# Autodesk Inventor assembly: !SCARA assembly
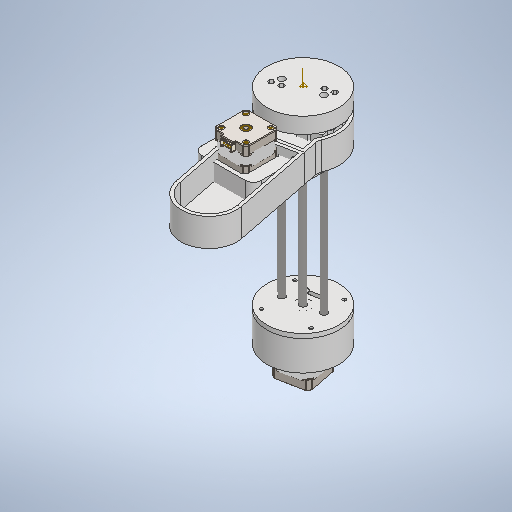
[picture p0: Inventor's stored thumbnail of the model, 512x512]
Saved by Autodesk Inventor 2025.2 (Build 292293000, 293)
## iProperties
Created: 2025-01-25
Part Number: !SCARA assembly
Document SubType Name: Assembly
Designer: caomi
Author: caomi
## Documents named in this file (18)
- C:\Minh Nguyen\H2A\cad\SCARA\!SCARA assembly.iam
- C:\Minh Nguyen\H2A\cad\SCARA\SCARA base.ipt
- C:\Minh Nguyen\H2A\cad\SCARA\Stepper Motor 17HS3401.ipt
- C:\Minh Nguyen\H2A\cad\SCARA\608 Bearing.ipt
- C:\Minh Nguyen\H2A\cad\SCARA\Shaft support.ipt
- C:\Minh Nguyen\H2A\cad\SCARA\SCARA swivel base - bottom.ipt
- C:\Minh Nguyen\H2A\cad\SCARA\Guide rods.ipt
- C:\Minh Nguyen\H2A\cad\SCARA\SCARA swivel base - mid.ipt
- C:\Minh Nguyen\H2A\cad\SCARA\Lead screw.ipt
- C:\Minh Nguyen\H2A\cad\SCARA\SCARA swivel connection rod.ipt
- C:\Minh Nguyen\H2A\cad\SCARA\Bearing block.ipt
- C:\Minh Nguyen\H2A\cad\SCARA\Lead nut.ipt
- C:\Minh Nguyen\H2A\cad\SCARA\SCARA arm base.ipt
- C:\Minh Nguyen\H2A\cad\SCARA\SCARA swivel top.ipt
- C:\Minh Nguyen\H2A\cad\SCARA\Shaft coupler.ipt
- C:\Minh Nguyen\H2A\cad\SCARA\SCARA arm.ipt
- C:\Minh Nguyen\H2A\cad\SCARA\SCARA swivel top - lid.ipt
- C:\Minh Nguyen\H2A\cad\SCARA\Limit_Switch.iam
## Components (24 placed, 17 different names)
1. SCARA base:1 — Slider:2, Rigid:1, Swivel base bottom - SCARA base
2. Stepper Motor 17HS3401:1 — Slider:2
3. 608 Bearing:1 — Rigid:1
4. SCARA swivel base - bottom:1 — Swivel base bottom - SCARA base, Swivel base mid - bottom, Swivel connection rod - swivel base bottom
5. SCARA swivel base - mid:1 — Swivel base mid - bottom, Support block 1 - Swivel base mid, Support block 2 - Swivel base mid, Bearing - Swivel base mid
6. Shaft support:1 — Support block 2 - Swivel base mid, Smooth rod 2 - Support block 2
7. Shaft support:2 — Support block 1 - Swivel base mid, Smooth rod 1 - Support block 1
8. 608 Bearing:2 — Bearing - Swivel base mid, Linear rod - Bearing
9. Guide rods:1 — Smooth rod 1 - Support block 1, Support block 3 - Smooth rod 1
10. Guide rods:2 — Smooth rod 2 - Support block 2, Smooth rods - SCARA arm base, Support block 4 - Smooth rod 1
11. Lead screw:1 — Linear rod - Bearing, Lead nut - Lead screw, Shaft coupler - Linear rod
12. SCARA swivel connection rod:1 — Swivel connection rod - swivel base bottom
13. Bearing block:1 — Support block 2 - SCARA arm base
14. Bearing block:2 — Support block 1 - SCARA arm base
15. Lead nut:1 — Lead nut - SCARA arm base, Lead nut - Lead screw
16. SCARA arm base:1 — Support block 1 - SCARA arm base, Support block 2 - SCARA arm base, Lead nut - SCARA arm base, Smooth rods - SCARA arm base, Swivel arm - Swivel arm base
17. Shaft support:3 — Support block 3 - Smooth rod 1, Swivel top - Support block 3
18. Shaft support:4 — Support block 4 - Smooth rod 1, Swivel top - Support block 4
19. SCARA swivel top:1 — Swivel top - Shaft coupler, Swivel top - Support block 3, Swivel top - Support block 4, Stepper motor - Shaft coupler, Swivel top - Swivel top lid, Limit Switch - Swivel top
20. Shaft coupler:1 — Shaft coupler - Linear rod, Swivel top - Shaft coupler
21. Stepper Motor 17HS3401:2 — Stepper motor - Shaft coupler
22. SCARA arm:1 — Swivel arm - Swivel arm base
23. SCARA swivel top - lid:1 — Swivel top - Swivel top lid
24. Limit_Switch:1 [sub-assembly] — Limit Switch - Swivel top
## Relationships (26: WeldJoint 19, RevoluteJoint 4, TranslationJoint 1, CylindricalJoint 1, Mate 1)
- Slider:2 [TranslationJoint]: SCARA base:1 ↔ Stepper Motor 17HS3401:1
- Rigid:1 [WeldJoint]: SCARA base:1 ↔ 608 Bearing:1
- Swivel base bottom - SCARA base [RevoluteJoint]: SCARA base:1 ↔ SCARA swivel base - bottom:1
- Swivel base mid - bottom [WeldJoint]: SCARA swivel base - bottom:1 ↔ SCARA swivel base - mid:1
- Support block 1 - Swivel base mid [WeldJoint]: SCARA swivel base - mid:1 ↔ Shaft support:2
- Support block 2 - Swivel base mid [WeldJoint]: SCARA swivel base - mid:1 ↔ Shaft support:1
- Bearing - Swivel base mid [WeldJoint]: SCARA swivel base - mid:1 ↔ 608 Bearing:2
- Smooth rod 1 - Support block 1 [WeldJoint]: Shaft support:2 ↔ Guide rods:1
- Smooth rod 2 - Support block 2 [WeldJoint]: Shaft support:1 ↔ Guide rods:2
- Linear rod - Bearing [WeldJoint]: 608 Bearing:2 ↔ Lead screw:1
- Support block 1 - SCARA arm base [WeldJoint]: Bearing block:2 ↔ SCARA arm base:1
- Support block 2 - SCARA arm base [WeldJoint]: Bearing block:1 ↔ SCARA arm base:1
- Lead nut - SCARA arm base [WeldJoint]: Lead nut:1 ↔ SCARA arm base:1
- Lead nut - Lead screw [CylindricalJoint]: Lead screw:1 ↔ Lead nut:1
- Smooth rods - SCARA arm base [Mate]: Guide rods:2 ↔ SCARA arm base:1
- Swivel connection rod - swivel base bottom [WeldJoint]: SCARA swivel base - bottom:1 ↔ SCARA swivel connection rod:1
- Support block 3 - Smooth rod 1 [RevoluteJoint]: Guide rods:1 ↔ Shaft support:3
- Support block 4 - Smooth rod 1 [RevoluteJoint]: Guide rods:2 ↔ Shaft support:4
- Shaft coupler - Linear rod [WeldJoint]: Lead screw:1 ↔ Shaft coupler:1
- Swivel top - Shaft coupler [RevoluteJoint]: SCARA swivel top:1 ↔ Shaft coupler:1
- Swivel top - Support block 3 [WeldJoint]: Shaft support:3 ↔ SCARA swivel top:1
- Swivel top - Support block 4 [WeldJoint]: Shaft support:4 ↔ SCARA swivel top:1
- Stepper motor - Shaft coupler [WeldJoint]: SCARA swivel top:1 ↔ Stepper Motor 17HS3401:2
- Swivel arm - Swivel arm base [WeldJoint]: SCARA arm base:1 ↔ SCARA arm:1
- Swivel top - Swivel top lid [WeldJoint]: SCARA swivel top:1 ↔ SCARA swivel top - lid:1
- Limit Switch - Swivel top [WeldJoint]: SCARA swivel top:1 ↔ Limit_Switch:1
